# Autodesk Inventor assembly: Backpack
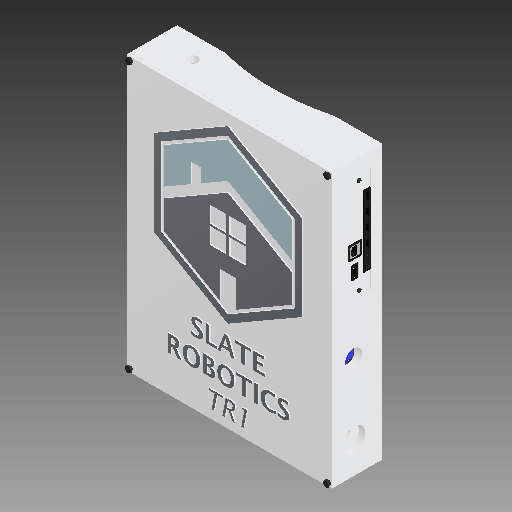
[picture p0: Inventor's stored thumbnail of the model, 512x512]
Saved by Autodesk Inventor 2017 SP1 (Build 210196100, 196)
## iProperties
Created: 2017-09-05
Part Number: Backpack
Document SubType Name: Assembly
Designer: Zach
Author: Zach
## Documents named in this file (26)
- C:\Users\Zach\Documents\GitHub\tr1\src\Body\Chest Assembly\Backpack Assembly\Backpack.iam
- C:\Users\Zach\Documents\GitHub\tr1\src\Body\Chest Assembly\Backpack Assembly\BP001b.ipt
- C:\Users\Zach\Documents\GitHub\tr1\src\Body\Chest Assembly\Backpack Assembly\BP002b.ipt
- C:\Users\Zach\Documents\GitHub\tr1\src\Body\Chest Assembly\Backpack Assembly\BP003.ipt
- C:\Users\Zach\Documents\GitHub\tr1\src\Body\Chest Assembly\Backpack Assembly\BP004.ipt
- C:\Users\Zach\Documents\GitHub\tr1\src\Body\Chest Assembly\Backpack Assembly\BP005.ipt
- C:\Users\Zach\Documents\GitHub\tr1\src\Body\Chest Assembly\Backpack Assembly\BP006.ipt
- C:\Users\Zach\Documents\GitHub\tr1\lib\Terminal Block 4\Клемная колодка ТВ-2504L 600V-25A\Клемная колодка ТВ-2504L 600V-25A.iam
- C:\Users\Zach\Documents\GitHub\tr1\lib\Arduino Nano\Arduino Nano V3 assemble.iam
- C:\Users\Zach\Documents\GitHub\tr1\lib\NVIDIA Jetson TK1\Jetson_TK1_FabD_3D.iam
- C:\Users\Zach\Documents\GitHub\tr1\lib\Arduino Mega 2560\Arduino Mega 2560.ipt
- C:\Users\Zach\Documents\GitHub\tr1\src\Body\Chest Assembly\Backpack Assembly\BP007.ipt
- C:\Users\Zach\Documents\GitHub\tr1\lib\L298n H Bridge\L298N\07j5423_1546306-8.ipt
- C:\Users\Zach\Documents\GitHub\tr1\lib\L298n Driver\l298n.ipt
- C:\Users\Zach\Documents\GitHub\tr1\src\Body\Chest Assembly\Backpack Assembly\BP008.ipt
- C:\Users\Zach\Documents\Inventor\Content Center Files\R2017\en-US\ISO 7045  H\ISO 7045 - M3 x 12 - 4.8 - H - ISO.ipt
- C:\Users\Zach\Documents\Inventor\Content Center Files\R2017\en-US\ISO 4035(2)\ISO 4035 - M5 - ISO.ipt
- C:\Users\Zach\Documents\Inventor\Content Center Files\R2017\en-US\ISO 4018\ISO 4018 - M5 x 25.ipt
- C:\Users\Zach\Documents\Inventor\Content Center Files\R2017\en-US\ISO 4018\ISO 4018 - M5 x 10.ipt
- C:\Users\Zach\Documents\GitHub\tr1\src\Body\Chest Assembly\Backpack Assembly\BP009.ipt
- C:\Users\Zach\Documents\GitHub\tr1\src\Body\Chest Assembly\Backpack Assembly\BP010.ipt
- C:\Users\Zach\Documents\GitHub\tr1\src\Body\Chest Assembly\Backpack Assembly\USB Hub.ipt
- C:\Users\Zach\Documents\GitHub\tr1\src\Body\Chest Assembly\Backpack Assembly\HDMI Port.ipt
- C:\Users\Zach\Documents\GitHub\tr1\src\Body\Chest Assembly\Backpack Assembly\Ethernet Port.ipt
- C:\Users\Zach\Documents\GitHub\tr1\src\Body\Chest Assembly\Backpack Assembly\SD Port.ipt
- C:\Users\Zach\Documents\Inventor\Content Center Files\R2017\en-US\ISO 4035(2)\ISO 4035 - M3 - ISO.ipt
## Components (132 placed, 25 different names)
1. BP001b:1 — Mate:1, Mate:2, Mate:3, Mate:6, Mate:8, Mate:9, Mate:11, Mate:13, Mate:15, Mate:19, Mate:20, Mate:21, Mate:22, Mate:23, Flush:1, Mate:24, Mate:25, Mate:26, Mate:35, Mate:36, Mate:37, Mate:38, Mate:39, Mate:42, Mate:43, Mate:44, Mate:45, Mate:46, Mate:56, Mate:57, Mate:58, Mate:78, Mate:79, Mate:80, Mate:81, Mate:82, Mate:133, Mate:134, Mate:137, Mate:138, Mate:141, Mate:142, Mate:145, Mate:146, Mate:149, Mate:150, Mate:160, Mate:161, Mate:162, Mate:163, Mate:176, Mate:177, Mate:178, Mate:179, Mate:180, Mate:181, Mate:182, Mate:183, Mate:184, Mate:185, Mate:186, Mate:187, Mate:188, Mate:189, Mate:190, Mate:191, Mate:196, Mate:200, Mate:201, Mate:202, Mate:203, Mate:270, Mate:271, Mate:272, Mate:280, Mate:310, Mate:312, Mate:314, Mate:316
2. BP002b:1 — Mate:1, Mate:2, Mate:3, Mate:204, Mate:205, Mate:206, Mate:207
3. BP003:1 — Mate:15, Mate:36, Mate:37, Mate:50, Mate:51, Mate:52, Mate:53, Mate:54, Mate:55, Mate:65, Angle:2, Mate:66, Mate:67, Mate:68, Mate:69, Mate:70, Mate:135, Mate:136, Mate:232, Mate:233, Mate:234, Mate:235, Mate:236, Mate:237, Mate:238, Mate:239, Mate:240, Mate:241, Mate:242, Mate:243, Mate:256, Mate:257, Mate:258
4. BP003:2 — Mate:19, Mate:27, Mate:28, Mate:29, Mate:30, Mate:31, Mate:32, Mate:38, Mate:39, Mate:59, Mate:60, Angle:1, Mate:61, Mate:62, Mate:63, Mate:64, Mate:139, Mate:140, Mate:208, Mate:209, Mate:210, Mate:211, Mate:212, Mate:213, Mate:214, Mate:215, Mate:216, Mate:217, Mate:218, Mate:219, Mate:259, Mate:260, Mate:261
5. BP004:1 — Mate:6, Mate:44, Mate:45, Mate:192, Mate:193, Mate:194, Mate:195, Mate:197, Mate:198, Mate:199
6. BP005:1 — Mate:8, Mate:9, Mate:20, Mate:172, Mate:173, Mate:174, Mate:175, Flush:9, Mate:287, Mate:288, Mate:307, Mate:308
7. BP006:1 — Mate:11, Mate:13, Mate:21, Mate:168, Mate:169, Mate:170, Mate:171, Flush:6, Mate:282, Mate:283, Flush:7, Mate:284, Mate:285, Flush:8, Mate:286
8. BP007:1 — Mate:46, Mate:75, Mate:76, Mate:77, Mate:78, Mate:79, Mate:87, Mate:88, Mate:89, Mate:94, Mate:95, Mate:100, Mate:111, Mate:112, Mate:113, Mate:114, Mate:115, Mate:293, Mate:296, Mate:297
9. BP007:2 — Mate:80, Mate:81, Mate:82, Mate:84, Mate:85, Mate:86, Mate:90, Mate:91, Mate:92, Mate:104, Mate:105, Mate:106, Mate:121, Mate:122, Mate:123, Mate:124, Mate:125, Mate:126, Mate:304, Mate:305, Mate:306
10. BP008:2 — Mate:87, Mate:88, Mate:89, Mate:93, Mate:97, Mate:98, Mate:99, Mate:101, Mate:102, Mate:289, Mate:290, Mate:291, Mate:292
11. BP008:3 — Mate:90, Mate:91, Mate:92, Mate:103, Mate:107, Mate:108, Mate:109, Mate:110, Mate:298, Mate:299, Mate:300, Mate:301
12. BP009:1 — Mate:256, Mate:257, Mate:258, Mate:264, Mate:265, Mate:266, Mate:267
13. BP009:2 — Mate:259, Mate:260, Mate:261, Mate:262, Mate:263, Mate:268, Mate:269
14. BP010:1 — Mate:270, Mate:271, Mate:272, Mate:273, Mate:274, Mate:275, Mate:276, Mate:277, Mate:278, Mate:279
15. Jetson_TK1_FabD_3D:1 [sub-assembly] — Mate:35, Mate:42, Mate:43, Mate:164, Mate:165, Mate:166, Mate:167
16. Клемная колодка ТВ-2504L 600V-25A:1 [sub-assembly] — Mate:24, Mate:25, Mate:26, Mate:151, Mate:152
17. Arduino Nano V3 assemble:1 [sub-assembly] — Mate:27, Mate:28, Mate:29
18. Arduino Nano V3 assemble:2 [sub-assembly] — Mate:30, Mate:31, Mate:32
19. Arduino Nano V3 assemble:3 [sub-assembly] — Mate:53, Mate:54, Mate:55
20. Arduino Nano V3 assemble:4 [sub-assembly] — Mate:50, Mate:51, Mate:52
21. Arduino Mega 2560:1 — Mate:75, Mate:76, Mate:77, Mate:96, Mate:116, Mate:117, Mate:118, Mate:119, Mate:120, Mate:293
22. Arduino Mega 2560:2 — Mate:84, Mate:85, Mate:86, Mate:127, Mate:128, Mate:129, Mate:130, Mate:131, Mate:132, Mate:306
23. 07j5423_1546306-8:1 — Mate:56, Mate:57, Mate:58, Mate:143, Mate:144, Mate:147, Mate:148
24. l298n:1 — Mate:59, Mate:60, Angle:1, Flush:3, Mate:228, Mate:229, Mate:230, Mate:231
25. l298n:2 — Mate:62, Mate:63, Flush:2, Flush:3, Mate:224, Mate:225, Mate:226, Mate:227
26. l298n:3 — Mate:61, Mate:64, Flush:2, Mate:220, Mate:221, Mate:222, Mate:223
27. l298n:4 — Mate:67, Mate:70, Flush:4, Flush:5, Mate:248, Mate:249, Mate:250, Mate:251
28. l298n:5 — Mate:68, Mate:69, Flush:5, Mate:252, Mate:253, Mate:254, Mate:255
29. l298n:6 — Mate:65, Angle:2, Mate:66, Flush:4, Mate:244, Mate:245, Mate:246, Mate:247
30. USB Hub:1 — Mate:280, Flush:6, Mate:286
31. HDMI Port:1 — Mate:282, Mate:283, Flush:7
32. Ethernet Port:1 — Mate:284, Mate:285, Flush:8
33. SD Port:1 — Flush:9, Mate:287, Mate:288
34. ISO 7045 H M3 x 12 - 4.8 - H:1 — Mate:95, Mate:96
35. ISO 4035 M5:1 — Mate:93, Mate:94
36. ISO 4018 M5 x 25:1 — Mate:97, Mate:98
37. ISO 4035 M5:2 — Mate:99, Mate:100
38. ISO 4018 M5 x 25:2 — Mate:101, Mate:102
39. ISO 4035 M5:3 — Mate:103, Mate:104
40. ISO 4035 M5:4 — Mate:105, Mate:106
41. ISO 4018 M5 x 25:3 — Mate:107, Mate:108
42. ISO 4018 M5 x 25:4 — Mate:109, Mate:110
43. ISO 7045 H M3 x 12 - 4.8 - H:2 — Mate:113, Mate:117
44. ISO 7045 H M3 x 12 - 4.8 - H:3 — Mate:112, Mate:119
45. ISO 7045 H M3 x 12 - 4.8 - H:4 — Mate:111, Mate:120
46. ISO 7045 H M3 x 12 - 4.8 - H:5 — Mate:114, Mate:118
47. ISO 7045 H M3 x 12 - 4.8 - H:6 — Mate:115, Mate:116
48. ISO 7045 H M3 x 12 - 4.8 - H:7 — Mate:121, Mate:128
49. ISO 7045 H M3 x 12 - 4.8 - H:8 — Mate:125, Mate:131
50. ISO 7045 H M3 x 12 - 4.8 - H:9 — Mate:126, Mate:132
51. ISO 7045 H M3 x 12 - 4.8 - H:10 — Mate:124, Mate:129
52. ISO 7045 H M3 x 12 - 4.8 - H:11 — Mate:122, Mate:130
53. ISO 7045 H M3 x 12 - 4.8 - H:12 — Mate:123, Mate:127
54. ISO 7045 H M3 x 12 - 4.8 - H:13 — Mate:133, Mate:136
55. ISO 7045 H M3 x 12 - 4.8 - H:14 — Mate:134, Mate:135
56. ISO 7045 H M3 x 12 - 4.8 - H:15 — Mate:137, Mate:139
57. ISO 7045 H M3 x 12 - 4.8 - H:16 — Mate:138, Mate:140
58. ISO 7045 H M3 x 12 - 4.8 - H:17 — Mate:142, Mate:143
59. ISO 7045 H M3 x 12 - 4.8 - H:18 — Mate:141, Mate:144
60. ISO 7045 H M3 x 12 - 4.8 - H:19 — Mate:146, Mate:148
61. ISO 7045 H M3 x 12 - 4.8 - H:20 — Mate:145, Mate:147
62. ISO 7045 H M3 x 12 - 4.8 - H:21 — Mate:149, Mate:152
63. ISO 7045 H M3 x 12 - 4.8 - H:22 — Mate:150, Mate:151
64. ISO 7045 H M3 x 12 - 4.8 - H:27 — Mate:160, Mate:165
65. ISO 7045 H M3 x 12 - 4.8 - H:28 — Mate:163, Mate:164
66. ISO 7045 H M3 x 12 - 4.8 - H:29 — Mate:161, Mate:166
67. ISO 7045 H M3 x 12 - 4.8 - H:30 — Mate:162, Mate:167
68. ISO 7045 H M3 x 12 - 4.8 - H:31 — Mate:169, Mate:170, Mate:313
69. ISO 7045 H M3 x 12 - 4.8 - H:32 — Mate:168, Mate:171, Mate:315
70. ISO 7045 H M3 x 12 - 4.8 - H:33 — Mate:172, Mate:173, Mate:309
71. ISO 7045 H M3 x 12 - 4.8 - H:34 — Mate:174, Mate:175
72. ISO 4018 M5 x 25:5 — Mate:179, Mate:190
73. ISO 4018 M5 x 25:6 — Mate:181, Mate:186
74. ISO 4018 M5 x 25:7 — Mate:182, Mate:187
75. ISO 4018 M5 x 25:8 — Mate:180, Mate:189
76. ISO 4018 M5 x 25:9 — Mate:177, Mate:191
77. ISO 4018 M5 x 25:10 — Mate:176, Mate:184
78. ISO 4018 M5 x 25:11 — Mate:178, Mate:185
79. ISO 4018 M5 x 25:12 — Mate:183, Mate:188
80. ISO 4018 M5 x 10:1 — Mate:192, Mate:193
81. ISO 4018 M5 x 10:3 — Mate:194, Mate:199
82. ISO 4018 M5 x 10:4 — Mate:196, Mate:197
83. ISO 4018 M5 x 10:5 — Mate:195, Mate:198
84. ISO 4018 M5 x 25:13 — Mate:200, Mate:205
85. ISO 4018 M5 x 25:14 — Mate:203, Mate:204
86. ISO 4018 M5 x 25:15 — Mate:202, Mate:207
87. ISO 4018 M5 x 25:16 — Mate:201, Mate:206
88. ISO 7045 H M3 x 12 - 4.8 - H:35 — Mate:219, Mate:230
89. ISO 7045 H M3 x 12 - 4.8 - H:36 — Mate:218, Mate:229
90. ISO 7045 H M3 x 12 - 4.8 - H:37 — Mate:217, Mate:228
91. ISO 7045 H M3 x 12 - 4.8 - H:38 — Mate:215, Mate:225
92. ISO 7045 H M3 x 12 - 4.8 - H:39 — Mate:216, Mate:231
93. ISO 7045 H M3 x 12 - 4.8 - H:40 — Mate:214, Mate:224
94. ISO 7045 H M3 x 12 - 4.8 - H:41 — Mate:213, Mate:226
95. ISO 7045 H M3 x 12 - 4.8 - H:42 — Mate:211, Mate:222
96. ISO 7045 H M3 x 12 - 4.8 - H:43 — Mate:210, Mate:223
97. ISO 7045 H M3 x 12 - 4.8 - H:44 — Mate:212, Mate:227
98. ISO 7045 H M3 x 12 - 4.8 - H:45 — Mate:209, Mate:220
99. ISO 7045 H M3 x 12 - 4.8 - H:46 — Mate:208, Mate:221
100. ISO 7045 H M3 x 12 - 4.8 - H:47 — Mate:238, Mate:248
101. ISO 7045 H M3 x 12 - 4.8 - H:48 — Mate:239, Mate:250
102. ISO 7045 H M3 x 12 - 4.8 - H:49 — Mate:243, Mate:254
103. ISO 7045 H M3 x 12 - 4.8 - H:50 — Mate:242, Mate:255
104. ISO 7045 H M3 x 12 - 4.8 - H:51 — Mate:232, Mate:245
105. ISO 7045 H M3 x 12 - 4.8 - H:52 — Mate:233, Mate:244
106. ISO 7045 H M3 x 12 - 4.8 - H:53 — Mate:235, Mate:246
107. ISO 7045 H M3 x 12 - 4.8 - H:54 — Mate:234, Mate:247
108. ISO 7045 H M3 x 12 - 4.8 - H:55 — Mate:236, Mate:249
109. ISO 7045 H M3 x 12 - 4.8 - H:56 — Mate:237, Mate:251
110. ISO 7045 H M3 x 12 - 4.8 - H:57 — Mate:240, Mate:253
111. ISO 7045 H M3 x 12 - 4.8 - H:58 — Mate:241, Mate:252
112. ISO 7045 H M3 x 12 - 4.8 - H:59 — Mate:262, Mate:269
113. ISO 7045 H M3 x 12 - 4.8 - H:60 — Mate:263, Mate:268
114. ISO 7045 H M3 x 12 - 4.8 - H:61 — Mate:264, Mate:267
115. ISO 7045 H M3 x 12 - 4.8 - H:62 — Mate:265, Mate:266
116. ISO 7045 H M3 x 12 - 4.8 - H:63 — Mate:273
117. ISO 7045 H M3 x 12 - 4.8 - H:64 — Mate:274, Mate:277
118. ISO 7045 H M3 x 12 - 4.8 - H:65 — Mate:275, Mate:278
119. ISO 7045 H M3 x 12 - 4.8 - H:66 — Mate:276, Mate:279
120. ISO 4018 M5 x 25:17 — Mate:291, Mate:292, Mate:295
121. ISO 4018 M5 x 25:18 — Mate:289, Mate:290, Mate:294
122. ISO 4035 M5:5 — Mate:294, Mate:297
123. ISO 4035 M5:6 — Mate:295, Mate:296
124. ISO 4018 M5 x 25:19 — Mate:299, Mate:300, Mate:302
125. ISO 4018 M5 x 25:20 — Mate:298, Mate:301, Mate:303
126. ISO 4035 M5:7 — Mate:302, Mate:305
127. ISO 4035 M5:8 — Mate:303, Mate:304
128. ISO 7045 H M3 x 12 - 4.8 - H:67 — Mate:307, Mate:308, Mate:311
129. ISO 4035 M3:1 — Mate:309, Mate:310
130. ISO 4035 M3:2 — Mate:311, Mate:312
131. ISO 4035 M3:3 — Mate:313, Mate:314
132. ISO 4035 M3:4 — Mate:315, Mate:316
## Relationships (298: Mate 287, Flush 9, Angle 2)
- Mate:1: BP001b:1 ↔ BP002b:1
- Mate:2: BP001b:1 ↔ BP002b:1
- Mate:3: BP001b:1 ↔ BP002b:1
- Mate:6: BP001b:1 ↔ BP004:1
- Mate:8: BP001b:1 ↔ BP005:1
- Mate:9: BP001b:1 ↔ BP005:1
- Mate:11: BP001b:1 ↔ BP006:1
- Mate:13: BP001b:1 ↔ BP006:1
- Mate:15: BP001b:1 ↔ BP003:1
- Mate:19: BP001b:1 ↔ BP003:2
- Mate:20: BP001b:1 ↔ BP005:1
- Mate:21: BP001b:1 ↔ BP006:1
- Mate:22: BP001b:1
- Mate:23: BP001b:1
- Flush:1 (200 mm): BP001b:1
- Mate:24: BP001b:1 ↔ Клемная колодка ТВ-2504L 600V-25A:1
- Mate:25: BP001b:1 ↔ Клемная колодка ТВ-2504L 600V-25A:1
- Mate:26: BP001b:1 ↔ Клемная колодка ТВ-2504L 600V-25A:1
- Mate:27: BP003:2 ↔ Arduino Nano V3 assemble:1
- Mate:28: BP003:2 ↔ Arduino Nano V3 assemble:1
- Mate:29 (0.6 mm): BP003:2 ↔ Arduino Nano V3 assemble:1
- Mate:30: BP003:2 ↔ Arduino Nano V3 assemble:2
- Mate:31: BP003:2 ↔ Arduino Nano V3 assemble:2
- Mate:32 (0.6 mm): BP003:2 ↔ Arduino Nano V3 assemble:2
- Mate:35: BP001b:1 ↔ Jetson_TK1_FabD_3D:1
- Mate:36: BP001b:1 ↔ BP003:1
- Mate:37: BP001b:1 ↔ BP003:1
- Mate:38: BP001b:1 ↔ BP003:2
- Mate:39: BP001b:1 ↔ BP003:2
- Mate:42: BP001b:1 ↔ Jetson_TK1_FabD_3D:1
- Mate:43: BP001b:1 ↔ Jetson_TK1_FabD_3D:1
- Mate:44: BP001b:1 ↔ BP004:1
- Mate:45: BP001b:1 ↔ BP004:1
- Mate:46: BP001b:1 ↔ BP007:1
- Mate:50: BP003:1 ↔ Arduino Nano V3 assemble:4
- Mate:51 (0.6 mm): BP003:1 ↔ Arduino Nano V3 assemble:4
- Mate:52: BP003:1 ↔ Arduino Nano V3 assemble:4
- Mate:53: BP003:1 ↔ Arduino Nano V3 assemble:3
- Mate:54 (0.6 mm): BP003:1 ↔ Arduino Nano V3 assemble:3
- Mate:55: BP003:1 ↔ Arduino Nano V3 assemble:3
- Mate:56: BP001b:1 ↔ 07j5423_1546306-8:1
- Mate:57: BP001b:1 ↔ 07j5423_1546306-8:1
- Mate:58: BP001b:1 ↔ 07j5423_1546306-8:1
- Mate:59: BP003:2 ↔ l298n:1
- Mate:60: BP003:2 ↔ l298n:1
- Angle:1 (180 deg): BP003:2 ↔ l298n:1
- Mate:61: BP003:2 ↔ l298n:3
- Mate:62: BP003:2 ↔ l298n:2
- Mate:63: BP003:2 ↔ l298n:2
- Mate:64: BP003:2 ↔ l298n:3
- Flush:2: l298n:2 ↔ l298n:3
- Flush:3: l298n:1 ↔ l298n:2
- Mate:65: BP003:1 ↔ l298n:6
- Angle:2 (180 deg): BP003:1 ↔ l298n:6
- Mate:66: BP003:1 ↔ l298n:6
- Mate:67: BP003:1 ↔ l298n:4
- Mate:68: BP003:1 ↔ l298n:5
- Mate:69: BP003:1 ↔ l298n:5
- Mate:70: BP003:1 ↔ l298n:4
- Flush:4: l298n:4 ↔ l298n:6
- Flush:5: l298n:4 ↔ l298n:5
- Mate:75: BP007:1 ↔ Arduino Mega 2560:1
- Mate:76: BP007:1 ↔ Arduino Mega 2560:1
- Mate:77: BP007:1 ↔ Arduino Mega 2560:1
- Mate:78: BP001b:1 ↔ BP007:1
- Mate:79: BP001b:1 ↔ BP007:1
- Mate:80: BP001b:1 ↔ BP007:2
- Mate:81: BP001b:1 ↔ BP007:2
- Mate:82: BP001b:1 ↔ BP007:2
- Mate:84: BP007:2 ↔ Arduino Mega 2560:2
- Mate:85: BP007:2 ↔ Arduino Mega 2560:2
- Mate:86: BP007:2 ↔ Arduino Mega 2560:2
- Mate:87: BP007:1 ↔ BP008:2
- Mate:88: BP007:1 ↔ BP008:2
- Mate:89: BP007:1 ↔ BP008:2
- Mate:90: BP007:2 ↔ BP008:3
- Mate:91: BP007:2 ↔ BP008:3
- Mate:92: BP007:2 ↔ BP008:3
- Mate:93: BP008:2 ↔ ISO 4035 M5:1
- Mate:94: BP007:1 ↔ ISO 4035 M5:1
- Mate:95: BP007:1 ↔ ISO 7045 H M3 x 12 - 4.8 - H:1
- Mate:96: Arduino Mega 2560:1 ↔ ISO 7045 H M3 x 12 - 4.8 - H:1
- Mate:97: BP008:2 ↔ ISO 4018 M5 x 25:1
- Mate:98: BP008:2 ↔ ISO 4018 M5 x 25:1
- Mate:99: BP008:2 ↔ ISO 4035 M5:2
- Mate:100: BP007:1 ↔ ISO 4035 M5:2
- Mate:101: BP008:2 ↔ ISO 4018 M5 x 25:2
- Mate:102: BP008:2 ↔ ISO 4018 M5 x 25:2
- Mate:103: BP008:3 ↔ ISO 4035 M5:3
- Mate:104: BP007:2 ↔ ISO 4035 M5:3
- Mate:105: BP007:2 ↔ ISO 4035 M5:4
- Mate:106: BP007:2 ↔ ISO 4035 M5:4
- Mate:107: BP008:3 ↔ ISO 4018 M5 x 25:3
- Mate:108: BP008:3 ↔ ISO 4018 M5 x 25:3
- Mate:109: BP008:3 ↔ ISO 4018 M5 x 25:4
- Mate:110: BP008:3 ↔ ISO 4018 M5 x 25:4
- Mate:111: BP007:1 ↔ ISO 7045 H M3 x 12 - 4.8 - H:4
- Mate:112: BP007:1 ↔ ISO 7045 H M3 x 12 - 4.8 - H:3
- Mate:113: BP007:1 ↔ ISO 7045 H M3 x 12 - 4.8 - H:2
- Mate:114: BP007:1 ↔ ISO 7045 H M3 x 12 - 4.8 - H:5
- Mate:115: BP007:1 ↔ ISO 7045 H M3 x 12 - 4.8 - H:6
- Mate:116: Arduino Mega 2560:1 ↔ ISO 7045 H M3 x 12 - 4.8 - H:6
- Mate:117: Arduino Mega 2560:1 ↔ ISO 7045 H M3 x 12 - 4.8 - H:2
- Mate:118: Arduino Mega 2560:1 ↔ ISO 7045 H M3 x 12 - 4.8 - H:5
- Mate:119: Arduino Mega 2560:1 ↔ ISO 7045 H M3 x 12 - 4.8 - H:3
- Mate:120: Arduino Mega 2560:1 ↔ ISO 7045 H M3 x 12 - 4.8 - H:4
- Mate:121: BP007:2 ↔ ISO 7045 H M3 x 12 - 4.8 - H:7
- Mate:122: BP007:2 ↔ ISO 7045 H M3 x 12 - 4.8 - H:11
- Mate:123: BP007:2 ↔ ISO 7045 H M3 x 12 - 4.8 - H:12
- Mate:124: BP007:2 ↔ ISO 7045 H M3 x 12 - 4.8 - H:10
- Mate:125: BP007:2 ↔ ISO 7045 H M3 x 12 - 4.8 - H:8
- Mate:126: BP007:2 ↔ ISO 7045 H M3 x 12 - 4.8 - H:9
- Mate:127: Arduino Mega 2560:2 ↔ ISO 7045 H M3 x 12 - 4.8 - H:12
- Mate:128: Arduino Mega 2560:2 ↔ ISO 7045 H M3 x 12 - 4.8 - H:7
- Mate:129: Arduino Mega 2560:2 ↔ ISO 7045 H M3 x 12 - 4.8 - H:10
- Mate:130: Arduino Mega 2560:2 ↔ ISO 7045 H M3 x 12 - 4.8 - H:11
- Mate:131: Arduino Mega 2560:2 ↔ ISO 7045 H M3 x 12 - 4.8 - H:8
- Mate:132: Arduino Mega 2560:2 ↔ ISO 7045 H M3 x 12 - 4.8 - H:9
- Mate:133: BP001b:1 ↔ ISO 7045 H M3 x 12 - 4.8 - H:13
- Mate:134: BP001b:1 ↔ ISO 7045 H M3 x 12 - 4.8 - H:14
- Mate:135: BP003:1 ↔ ISO 7045 H M3 x 12 - 4.8 - H:14
- Mate:136: BP003:1 ↔ ISO 7045 H M3 x 12 - 4.8 - H:13
- Mate:137: BP001b:1 ↔ ISO 7045 H M3 x 12 - 4.8 - H:15
- Mate:138: BP001b:1 ↔ ISO 7045 H M3 x 12 - 4.8 - H:16
- Mate:139: BP003:2 ↔ ISO 7045 H M3 x 12 - 4.8 - H:15
- Mate:140: BP003:2 ↔ ISO 7045 H M3 x 12 - 4.8 - H:16
- Mate:141: BP001b:1 ↔ ISO 7045 H M3 x 12 - 4.8 - H:18
- Mate:142: BP001b:1 ↔ ISO 7045 H M3 x 12 - 4.8 - H:17
- Mate:143: 07j5423_1546306-8:1 ↔ ISO 7045 H M3 x 12 - 4.8 - H:17
- Mate:144: 07j5423_1546306-8:1 ↔ ISO 7045 H M3 x 12 - 4.8 - H:18
- Mate:145: BP001b:1 ↔ ISO 7045 H M3 x 12 - 4.8 - H:20
- Mate:146: BP001b:1 ↔ ISO 7045 H M3 x 12 - 4.8 - H:19
- Mate:147: 07j5423_1546306-8:1 ↔ ISO 7045 H M3 x 12 - 4.8 - H:20
- Mate:148: 07j5423_1546306-8:1 ↔ ISO 7045 H M3 x 12 - 4.8 - H:19
- Mate:149: BP001b:1 ↔ ISO 7045 H M3 x 12 - 4.8 - H:21
- Mate:150: BP001b:1 ↔ ISO 7045 H M3 x 12 - 4.8 - H:22
- Mate:151: Клемная колодка ТВ-2504L 600V-25A:1 ↔ ISO 7045 H M3 x 12 - 4.8 - H:22
- Mate:152: Клемная колодка ТВ-2504L 600V-25A:1 ↔ ISO 7045 H M3 x 12 - 4.8 - H:21
- Mate:160: BP001b:1 ↔ ISO 7045 H M3 x 12 - 4.8 - H:27
- Mate:161: BP001b:1 ↔ ISO 7045 H M3 x 12 - 4.8 - H:29
- Mate:162: BP001b:1 ↔ ISO 7045 H M3 x 12 - 4.8 - H:30
- Mate:163: BP001b:1 ↔ ISO 7045 H M3 x 12 - 4.8 - H:28
- Mate:164: Jetson_TK1_FabD_3D:1 ↔ ISO 7045 H M3 x 12 - 4.8 - H:28
- Mate:165: Jetson_TK1_FabD_3D:1 ↔ ISO 7045 H M3 x 12 - 4.8 - H:27
- Mate:166: Jetson_TK1_FabD_3D:1 ↔ ISO 7045 H M3 x 12 - 4.8 - H:29
- Mate:167: Jetson_TK1_FabD_3D:1 ↔ ISO 7045 H M3 x 12 - 4.8 - H:30
- Mate:168: BP006:1 ↔ ISO 7045 H M3 x 12 - 4.8 - H:32
- Mate:169: BP006:1 ↔ ISO 7045 H M3 x 12 - 4.8 - H:31
- Mate:170: BP006:1 ↔ ISO 7045 H M3 x 12 - 4.8 - H:31
- Mate:171: BP006:1 ↔ ISO 7045 H M3 x 12 - 4.8 - H:32
- Mate:172: BP005:1 ↔ ISO 7045 H M3 x 12 - 4.8 - H:33
- Mate:173: BP005:1 ↔ ISO 7045 H M3 x 12 - 4.8 - H:33
- Mate:174: BP005:1 ↔ ISO 7045 H M3 x 12 - 4.8 - H:34
- Mate:175: BP005:1 ↔ ISO 7045 H M3 x 12 - 4.8 - H:34
- Mate:176: BP001b:1 ↔ ISO 4018 M5 x 25:10
- Mate:177: BP001b:1 ↔ ISO 4018 M5 x 25:9
- Mate:178: BP001b:1 ↔ ISO 4018 M5 x 25:11
- Mate:179: BP001b:1 ↔ ISO 4018 M5 x 25:5
- Mate:180: BP001b:1 ↔ ISO 4018 M5 x 25:8
- Mate:181: BP001b:1 ↔ ISO 4018 M5 x 25:6
- Mate:182: BP001b:1 ↔ ISO 4018 M5 x 25:7
- Mate:183: BP001b:1 ↔ ISO 4018 M5 x 25:12
- Mate:184: BP001b:1 ↔ ISO 4018 M5 x 25:10
- Mate:185: BP001b:1 ↔ ISO 4018 M5 x 25:11
- Mate:186: BP001b:1 ↔ ISO 4018 M5 x 25:6
- Mate:187: BP001b:1 ↔ ISO 4018 M5 x 25:7
- Mate:188: BP001b:1 ↔ ISO 4018 M5 x 25:12
- Mate:189: BP001b:1 ↔ ISO 4018 M5 x 25:8
- Mate:190: BP001b:1 ↔ ISO 4018 M5 x 25:5
- Mate:191: BP001b:1 ↔ ISO 4018 M5 x 25:9
- Mate:192: BP004:1 ↔ ISO 4018 M5 x 10:1
- Mate:193: BP004:1 ↔ ISO 4018 M5 x 10:1
- Mate:194: BP004:1 ↔ ISO 4018 M5 x 10:3
- Mate:195: BP004:1 ↔ ISO 4018 M5 x 10:5
- Mate:196: BP001b:1 ↔ ISO 4018 M5 x 10:4
- Mate:197: BP004:1 ↔ ISO 4018 M5 x 10:4
- Mate:198: BP004:1 ↔ ISO 4018 M5 x 10:5
- Mate:199: BP004:1 ↔ ISO 4018 M5 x 10:3
- Mate:200: BP001b:1 ↔ ISO 4018 M5 x 25:13
- Mate:201: BP001b:1 ↔ ISO 4018 M5 x 25:16
- Mate:202: BP001b:1 ↔ ISO 4018 M5 x 25:15
- Mate:203: BP001b:1 ↔ ISO 4018 M5 x 25:14
- Mate:204: BP002b:1 ↔ ISO 4018 M5 x 25:14
- Mate:205: BP002b:1 ↔ ISO 4018 M5 x 25:13
- Mate:206: BP002b:1 ↔ ISO 4018 M5 x 25:16
- Mate:207: BP002b:1 ↔ ISO 4018 M5 x 25:15
- Mate:208: BP003:2 ↔ ISO 7045 H M3 x 12 - 4.8 - H:46
- Mate:209: BP003:2 ↔ ISO 7045 H M3 x 12 - 4.8 - H:45
- Mate:210: BP003:2 ↔ ISO 7045 H M3 x 12 - 4.8 - H:43
- Mate:211: BP003:2 ↔ ISO 7045 H M3 x 12 - 4.8 - H:42
- Mate:212: BP003:2 ↔ ISO 7045 H M3 x 12 - 4.8 - H:44
- Mate:213: BP003:2 ↔ ISO 7045 H M3 x 12 - 4.8 - H:41
- Mate:214: BP003:2 ↔ ISO 7045 H M3 x 12 - 4.8 - H:40
- Mate:215: BP003:2 ↔ ISO 7045 H M3 x 12 - 4.8 - H:38
- Mate:216: BP003:2 ↔ ISO 7045 H M3 x 12 - 4.8 - H:39
- Mate:217: BP003:2 ↔ ISO 7045 H M3 x 12 - 4.8 - H:37
- Mate:218: BP003:2 ↔ ISO 7045 H M3 x 12 - 4.8 - H:36
- Mate:219: BP003:2 ↔ ISO 7045 H M3 x 12 - 4.8 - H:35
- Mate:220: l298n:3 ↔ ISO 7045 H M3 x 12 - 4.8 - H:45
- Mate:221: l298n:3 ↔ ISO 7045 H M3 x 12 - 4.8 - H:46
- Mate:222: l298n:3 ↔ ISO 7045 H M3 x 12 - 4.8 - H:42
- Mate:223: l298n:3 ↔ ISO 7045 H M3 x 12 - 4.8 - H:43
- Mate:224: l298n:2 ↔ ISO 7045 H M3 x 12 - 4.8 - H:40
- Mate:225: l298n:2 ↔ ISO 7045 H M3 x 12 - 4.8 - H:38
- Mate:226: l298n:2 ↔ ISO 7045 H M3 x 12 - 4.8 - H:41
- Mate:227: l298n:2 ↔ ISO 7045 H M3 x 12 - 4.8 - H:44
- Mate:228: l298n:1 ↔ ISO 7045 H M3 x 12 - 4.8 - H:37
- Mate:229: l298n:1 ↔ ISO 7045 H M3 x 12 - 4.8 - H:36
- Mate:230: l298n:1 ↔ ISO 7045 H M3 x 12 - 4.8 - H:35
- Mate:231: l298n:1 ↔ ISO 7045 H M3 x 12 - 4.8 - H:39
- Mate:232: BP003:1 ↔ ISO 7045 H M3 x 12 - 4.8 - H:51
- Mate:233: BP003:1 ↔ ISO 7045 H M3 x 12 - 4.8 - H:52
- Mate:234: BP003:1 ↔ ISO 7045 H M3 x 12 - 4.8 - H:54
- Mate:235: BP003:1 ↔ ISO 7045 H M3 x 12 - 4.8 - H:53
- Mate:236: BP003:1 ↔ ISO 7045 H M3 x 12 - 4.8 - H:55
- Mate:237: BP003:1 ↔ ISO 7045 H M3 x 12 - 4.8 - H:56
- Mate:238: BP003:1 ↔ ISO 7045 H M3 x 12 - 4.8 - H:47
- Mate:239: BP003:1 ↔ ISO 7045 H M3 x 12 - 4.8 - H:48
- Mate:240: BP003:1 ↔ ISO 7045 H M3 x 12 - 4.8 - H:57
- Mate:241: BP003:1 ↔ ISO 7045 H M3 x 12 - 4.8 - H:58
- Mate:242: BP003:1 ↔ ISO 7045 H M3 x 12 - 4.8 - H:50
- Mate:243: BP003:1 ↔ ISO 7045 H M3 x 12 - 4.8 - H:49
- Mate:244: l298n:6 ↔ ISO 7045 H M3 x 12 - 4.8 - H:52
- Mate:245: l298n:6 ↔ ISO 7045 H M3 x 12 - 4.8 - H:51
- Mate:246: l298n:6 ↔ ISO 7045 H M3 x 12 - 4.8 - H:53
- Mate:247: l298n:6 ↔ ISO 7045 H M3 x 12 - 4.8 - H:54
- Mate:248: l298n:4 ↔ ISO 7045 H M3 x 12 - 4.8 - H:47
- Mate:249: l298n:4 ↔ ISO 7045 H M3 x 12 - 4.8 - H:55
- Mate:250: l298n:4 ↔ ISO 7045 H M3 x 12 - 4.8 - H:48
- Mate:251: l298n:4 ↔ ISO 7045 H M3 x 12 - 4.8 - H:56
- Mate:252: l298n:5 ↔ ISO 7045 H M3 x 12 - 4.8 - H:58
- Mate:253: l298n:5 ↔ ISO 7045 H M3 x 12 - 4.8 - H:57
- Mate:254: l298n:5 ↔ ISO 7045 H M3 x 12 - 4.8 - H:49
- Mate:255: l298n:5 ↔ ISO 7045 H M3 x 12 - 4.8 - H:50
- Mate:256: BP003:1 ↔ BP009:1
- Mate:257: BP003:1 ↔ BP009:1
- Mate:258: BP003:1 ↔ BP009:1
- Mate:259: BP003:2 ↔ BP009:2
- Mate:260: BP003:2 ↔ BP009:2
- Mate:261: BP003:2 ↔ BP009:2
- Mate:262: BP009:2 ↔ ISO 7045 H M3 x 12 - 4.8 - H:59
- Mate:263: BP009:2 ↔ ISO 7045 H M3 x 12 - 4.8 - H:60
- Mate:264: BP009:1 ↔ ISO 7045 H M3 x 12 - 4.8 - H:61
- Mate:265: BP009:1 ↔ ISO 7045 H M3 x 12 - 4.8 - H:62
- Mate:266: BP009:1 ↔ ISO 7045 H M3 x 12 - 4.8 - H:62
- Mate:267: BP009:1 ↔ ISO 7045 H M3 x 12 - 4.8 - H:61
- Mate:268: BP009:2 ↔ ISO 7045 H M3 x 12 - 4.8 - H:60
- Mate:269: BP009:2 ↔ ISO 7045 H M3 x 12 - 4.8 - H:59
- Mate:270: BP001b:1 ↔ BP010:1
- Mate:271: BP001b:1 ↔ BP010:1
- Mate:272: BP001b:1 ↔ BP010:1
- Mate:273: BP010:1 ↔ ISO 7045 H M3 x 12 - 4.8 - H:63
- Mate:274: BP010:1 ↔ ISO 7045 H M3 x 12 - 4.8 - H:64
- Mate:275: BP010:1 ↔ ISO 7045 H M3 x 12 - 4.8 - H:65
- Mate:276: BP010:1 ↔ ISO 7045 H M3 x 12 - 4.8 - H:66
- Mate:277: BP010:1 ↔ ISO 7045 H M3 x 12 - 4.8 - H:64
- Mate:278: BP010:1 ↔ ISO 7045 H M3 x 12 - 4.8 - H:65
- Mate:279: BP010:1 ↔ ISO 7045 H M3 x 12 - 4.8 - H:66
- Mate:280: BP001b:1 ↔ USB Hub:1
- Flush:6: BP006:1 ↔ USB Hub:1
- Mate:282 (0.5 mm): BP006:1 ↔ HDMI Port:1
- Mate:283 (0.5 mm): BP006:1 ↔ HDMI Port:1
- Flush:7: BP006:1 ↔ HDMI Port:1
- Mate:284: BP006:1 ↔ Ethernet Port:1
- Mate:285 (0.5 mm): BP006:1 ↔ Ethernet Port:1
- Flush:8: BP006:1 ↔ Ethernet Port:1
- Mate:286 (0.5 mm): BP006:1 ↔ USB Hub:1
- Flush:9: BP005:1 ↔ SD Port:1
- Mate:287 (0.5 mm): BP005:1 ↔ SD Port:1
- Mate:288 (0.5 mm): BP005:1 ↔ SD Port:1
- Mate:289: BP008:2 ↔ ISO 4018 M5 x 25:18
- Mate:290: BP008:2 ↔ ISO 4018 M5 x 25:18
- Mate:291: BP008:2 ↔ ISO 4018 M5 x 25:17
- Mate:292: BP008:2 ↔ ISO 4018 M5 x 25:17
- Mate:293: BP007:1 ↔ Arduino Mega 2560:1
- Mate:294: ISO 4018 M5 x 25:18 ↔ ISO 4035 M5:5
- Mate:295: ISO 4018 M5 x 25:17 ↔ ISO 4035 M5:6
- Mate:296: BP007:1 ↔ ISO 4035 M5:6
- Mate:297: BP007:1 ↔ ISO 4035 M5:5
- Mate:298: BP008:3 ↔ ISO 4018 M5 x 25:20
- Mate:299: BP008:3 ↔ ISO 4018 M5 x 25:19
- Mate:300: BP008:3 ↔ ISO 4018 M5 x 25:19
- Mate:301: BP008:3 ↔ ISO 4018 M5 x 25:20
- Mate:302: ISO 4018 M5 x 25:19 ↔ ISO 4035 M5:7
- Mate:303: ISO 4018 M5 x 25:20 ↔ ISO 4035 M5:8
- Mate:304: BP007:2 ↔ ISO 4035 M5:8
- Mate:305: BP007:2 ↔ ISO 4035 M5:7
- Mate:306: BP007:2 ↔ Arduino Mega 2560:2
- Mate:307: BP005:1 ↔ ISO 7045 H M3 x 12 - 4.8 - H:67
- Mate:308: BP005:1 ↔ ISO 7045 H M3 x 12 - 4.8 - H:67
- Mate:309: ISO 7045 H M3 x 12 - 4.8 - H:33 ↔ ISO 4035 M3:1
- Mate:310: BP001b:1 ↔ ISO 4035 M3:1
- Mate:311: ISO 7045 H M3 x 12 - 4.8 - H:67 ↔ ISO 4035 M3:2
- Mate:312: BP001b:1 ↔ ISO 4035 M3:2
- Mate:313: ISO 7045 H M3 x 12 - 4.8 - H:31 ↔ ISO 4035 M3:3
- Mate:314: BP001b:1 ↔ ISO 4035 M3:3
- Mate:315: ISO 7045 H M3 x 12 - 4.8 - H:32 ↔ ISO 4035 M3:4
- Mate:316: BP001b:1 ↔ ISO 4035 M3:4
